# Autodesk Inventor assembly: Garage_roof_side
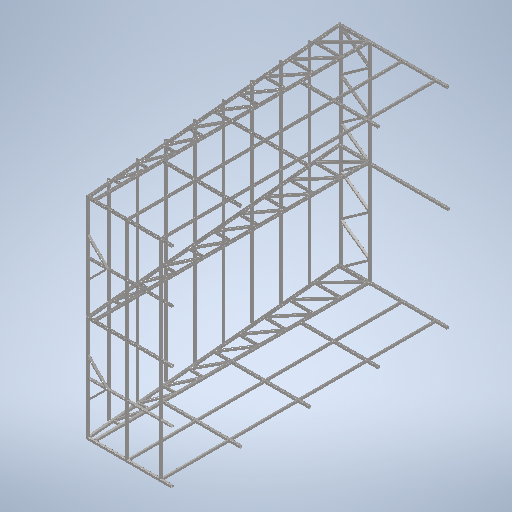
[picture p0: Inventor's stored thumbnail of the model, 512x512]
Saved by Autodesk Inventor 2025.2 (Build 292293000, 293)
## iProperties
Created: 2025-09-27
Part Number: Garage_roof_side
Document SubType Name: Assembly
Designer: MB
Mass: 921925 g
Surface Area: 837843 cm^2
Volume: 117443 cm^3
Density: 7.85 g/cm^3
_SolveAssemblyDoc: Frame Generator Solve Assembly
_Version: 25.0.0
Author: MB
## Documents named in this file (3)
- C:\Users\MB\Documents\GitHub\hegesztes\Garage_roof_side.iam
- C:\Users\MB\Documents\GitHub\hegesztes\Roof_side_left.ipt
- C:\Users\MB\Documents\GitHub\hegesztes\Garage_roof_side\Frame\Frame 1759007616013.iam
## Components (2 placed, 2 different names)
1. Roof_side_left:1 — Flush:1, Flush:3, Flush:5
2. Frame 1759007616013:1 [sub-assembly] — Flush:1, Flush:2, Flush:3, Flush:4
## Relationships (5: Flush 5)
- Flush:1: Roof_side_left:1 ↔ Frame 1759007616013:1
- Flush:2 (-30 mm): Frame 1759007616013:1
- Flush:3 (-30 mm): Roof_side_left:1 ↔ Frame 1759007616013:1
- Flush:4 (30 mm): Frame 1759007616013:1
- Flush:5: Roof_side_left:1
